# Autodesk Inventor assembly: FRCIntake2024
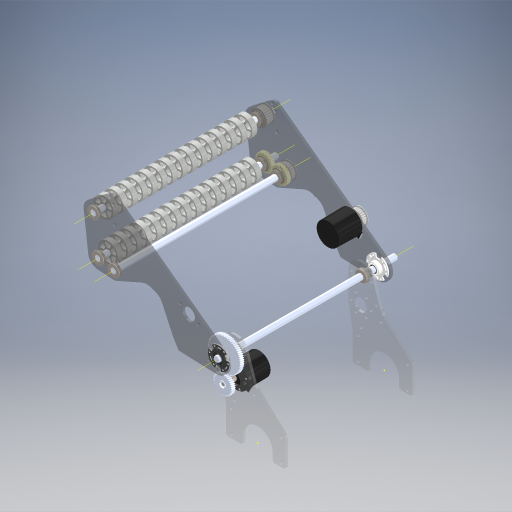
[picture p0: Inventor's stored thumbnail of the model, 512x512]
Saved by Autodesk Inventor 2024.2 (Build 282272000, 272)
## iProperties
Created: 2024-02-17
Part Number: FRCIntake2024
Document SubType Name: Assembly
Designer: rohan
Mass: 2142.23 g
Surface Area: 6813.45 cm^2
Volume: 1719.02 cm^3
Density: 1.24619 g/cm^3
Author: rohan
## Documents named in this file (14)
- C:\Users\rohan\OneDrive - Hillsborough County Public Schools\Robotics\FIRST-Robotics-Competition\Crescendo\Minotaur-Crescendo-Robot\FRCIntake2024.iam
- C:\Users\rohan\OneDrive - Hillsborough County Public Schools\Robotics\FIRST-Robotics-Competition\Crescendo\Minotaur-Crescendo-Robot\2D Overview - Part 2\wfsdf.ipt
- C:\Users\rohan\OneDrive - Hillsborough County Public Schools\Robotics\FIRST-Robotics-Competition\Crescendo\Minotaur-Crescendo-Robot\2D Overview - Part 2\cranking90s.ipt
- C:\Users\rohan\OneDrive - Hillsborough County Public Schools\Robotics\FIRST-Robotics-Competition\Crescendo\Minotaur-Crescendo-Robot\2D Overview - Part 2\am-2986 FR8ZZ Hex Bearing.ipt
- C:\Users\rohan\OneDrive - Hillsborough County Public Schools\Robotics\FIRST-Robotics-Competition\Crescendo\Minotaur-Crescendo-Robot\2D Overview - Part 2\1_2 Hex Bore Plastic VersaHub v2 (217-8079).iam
- C:\Users\rohan\OneDrive - Hillsborough County Public Schools\Robotics\FIRST-Robotics-Competition\Crescendo\Minotaur-Crescendo-Robot\2D Overview - Part 2\1_2 Acetal Spacer - 1_2 Hex (217-3261).ipt
- C:\Users\rohan\OneDrive - Hillsborough County Public Schools\Robotics\FIRST-Robotics-Competition\Crescendo\Minotaur-Crescendo-Robot\2D Overview - Part 2\1_2 OD Hex Stock (18) (217-3309).ipt
- C:\Users\rohan\Downloads\Minotaur-2024-CAD-main (2)\Minotaur-2024-CAD-main\Minotaur-2024-CAD-main\Minotaur-2024-CAD-main\64T Aluminum Spur Gear (20 DP, 1_2 Hex Bore) (217-3575)\64T Aluminum Spur Gear (20 DP, 1_.ipt
- C:\Users\rohan\Downloads\Minotaur-2024-CAD-main (2)\Minotaur-2024-CAD-main\Minotaur-2024-CAD-main\Minotaur-2024-CAD-main\Electronics\NEO-Brushless-Motor.ipt
- C:\Users\rohan\Downloads\36T Aluminum Spur Gear (20 DP, 1_2 Hex Bore) (217-3214)\36T Aluminum Spur Gear (20 DP, 1_2 Hex Bore) (217-3214).ipt
- C:\Users\rohan\OneDrive - Hillsborough County Public Schools\Robotics\FIRST-Robotics-Competition\Crescendo\Minotaur-Crescendo-Robot\2D Overview - Part 2\2 OD Straight Flex Wheel (217-6353).ipt
- C:\Users\rohan\OneDrive - Hillsborough County Public Schools\Robotics\FIRST-Robotics-Competition\Crescendo\Minotaur-Crescendo-Robot\2D Overview - Part 2\24t 15mm Wide 1_2_ Hex Bore Double Flange 5mm HTD Aluminum Pulley (217-4101).ipt
- C:\Users\rohan\OneDrive - Hillsborough County Public Schools\Robotics\FIRST-Robotics-Competition\Crescendo\Minotaur-Crescendo-Robot\2D Overview - Part 2\32t 20dp Aluminum 1_2_ Hex Bore Gear (217-5470).ipt
- C:\Users\rohan\OneDrive - Hillsborough County Public Schools\Robotics\FIRST-Robotics-Competition\Crescendo\Minotaur-Crescendo-Robot\2D Overview - Part 2\24t 9mm Wide 1_2_ Hex Bore Double Flange 5mm HTD Aluminum Pulley (217-3227).ipt
## Components (59 placed, 13 different names)
1. wfsdf:1 — Mate:1, Flush:1, Flush:2, Insert:2, Mate:8
2. wfsdf:2 — Mate:1, Flush:1, Flush:2, Insert:1, Mate:13, Mate:14
3. cranking90s:1 — Mate:11, Flush:3, Insert:8, Insert:9, Insert:10, Mate:16, Mate:20, Flush:7, Mate:26
4. cranking90s:2 — Mate:9, Mate:10, Flush:3, Insert:5, Insert:6, Insert:7, Mate:17, Mate:18, Mate:23, Mate:24
5. am-2986 FR8ZZ Hex Bearing:1 — Insert:2, Mate:2, Mate:6
6. am-2986 FR8ZZ Hex Bearing:2 — Insert:1, Mate:4
7. 1_2 Hex Bore Plastic VersaHub v2 (217-8079):1 [sub-assembly] — Mate:7, Mate:8, Mate:10
8. 1_2 Hex Bore Plastic VersaHub v2 (217-8079):2 [sub-assembly] — Mate:25, Mate:26
9. 1_2 Acetal Spacer - 1_2 Hex (217-3261):1 — Mate:3, Mate:4, Insert:3
10. 1_2 Acetal Spacer - 1_2 Hex (217-3261):2 — Mate:5, Mate:6
11. 1_2 OD Hex Stock (18) (217-3309):1 — Mate:2, Mate:3, Mate:5, Mate:7, Mate:9, Mate:11, Flush:7, Mate:25
12. 64T Aluminum Spur Gear (20 DP, 1_:1 — Insert:3
13. NEO-Brushless-Motor:1 — Mate:13, Mate:14, Insert:4
14. 36T Aluminum Spur Gear (20 DP, 1_2 Hex Bore) (217-3214):1 — Insert:4
15. am-2986 FR8ZZ Hex Bearing:3 — Insert:7, Insert:13
16. am-2986 FR8ZZ Hex Bearing:4 — Insert:10, Flush:5
17. am-2986 FR8ZZ Hex Bearing:5 — Insert:9, Flush:6, Mate:22
18. am-2986 FR8ZZ Hex Bearing:6 — Insert:6, Insert:12
19. am-2986 FR8ZZ Hex Bearing:7 — Insert:8, Flush:4
20. am-2986 FR8ZZ Hex Bearing:8 — Insert:5, Insert:11
21. 1_2 OD Hex Stock (18) (217-3309):2 — Mate:16, Flush:4, Mate:19
22. 1_2 OD Hex Stock (18) (217-3309):3 — Mate:17, Flush:5
23. 1_2 OD Hex Stock (18) (217-3309):4 — Mate:18, Flush:6, Mate:21
24. 24t 15mm Wide 1_2_ Hex Bore Double Flange 5mm HTD Aluminum Pulley (217-4101):1 — Insert:11
25. 32t 20dp Aluminum 1_2_ Hex Bore Gear (217-5470):1 — Insert:13, Insert:14
26. 32t 20dp Aluminum 1_2_ Hex Bore Gear (217-5470):2 — Insert:12
27. 24t 9mm Wide 1_2_ Hex Bore Double Flange 5mm HTD Aluminum Pulley (217-3227):1 — Insert:14
28. NEO-Brushless-Motor:2 — Mate:23, Mate:24, Insert:15
29. 24t 9mm Wide 1_2_ Hex Bore Double Flange 5mm HTD Aluminum Pulley (217-3227):2 — Insert:15
30. 2 OD Straight Flex Wheel (217-6353):1 — Mate:19, Mate:20
31. 2 OD Straight Flex Wheel (217-6353):2
32. 2 OD Straight Flex Wheel (217-6353):3
33. 2 OD Straight Flex Wheel (217-6353):4
34. 2 OD Straight Flex Wheel (217-6353):5
35. 2 OD Straight Flex Wheel (217-6353):6
36. 2 OD Straight Flex Wheel (217-6353):7
37. 2 OD Straight Flex Wheel (217-6353):8
38. 2 OD Straight Flex Wheel (217-6353):9
39. 2 OD Straight Flex Wheel (217-6353):10
40. 2 OD Straight Flex Wheel (217-6353):11
41. 2 OD Straight Flex Wheel (217-6353):12
42. 2 OD Straight Flex Wheel (217-6353):13
43. 2 OD Straight Flex Wheel (217-6353):14
44. 2 OD Straight Flex Wheel (217-6353):15
45. 2 OD Straight Flex Wheel (217-6353):16 — Mate:21, Mate:22
46. 2 OD Straight Flex Wheel (217-6353):17
47. 2 OD Straight Flex Wheel (217-6353):18
48. 2 OD Straight Flex Wheel (217-6353):19
49. 2 OD Straight Flex Wheel (217-6353):20
50. 2 OD Straight Flex Wheel (217-6353):21
51. 2 OD Straight Flex Wheel (217-6353):22
52. 2 OD Straight Flex Wheel (217-6353):23
53. 2 OD Straight Flex Wheel (217-6353):24
54. 2 OD Straight Flex Wheel (217-6353):25
55. 2 OD Straight Flex Wheel (217-6353):26
56. 2 OD Straight Flex Wheel (217-6353):27
57. 2 OD Straight Flex Wheel (217-6353):28
58. 2 OD Straight Flex Wheel (217-6353):29
59. 2 OD Straight Flex Wheel (217-6353):30
## Component patterns: (15 elements, first: 2 OD Straight Flex Wheel (217-6353):1), (15 elements, first: 2 OD Straight Flex Wheel (217-6353):16)
## Relationships (46: Mate 24, Insert 15, Flush 7)
- Mate:1 (317.5 mm): wfsdf:1 ↔ wfsdf:2
- Flush:1: wfsdf:1 ↔ wfsdf:2
- Flush:2: wfsdf:1 ↔ wfsdf:2
- Insert:1: wfsdf:2 ↔ am-2986 FR8ZZ Hex Bearing:2
- Insert:2: wfsdf:1 ↔ am-2986 FR8ZZ Hex Bearing:1
- Mate:2: am-2986 FR8ZZ Hex Bearing:1 ↔ 1_2 OD Hex Stock (18) (217-3309):1
- Mate:3: 1_2 Acetal Spacer - 1_2 Hex (217-3261):1 ↔ 1_2 OD Hex Stock (18) (217-3309):1
- Mate:4: am-2986 FR8ZZ Hex Bearing:2 ↔ 1_2 Acetal Spacer - 1_2 Hex (217-3261):1
- Mate:5: 1_2 Acetal Spacer - 1_2 Hex (217-3261):2 ↔ 1_2 OD Hex Stock (18) (217-3309):1
- Mate:6: am-2986 FR8ZZ Hex Bearing:1 ↔ 1_2 Acetal Spacer - 1_2 Hex (217-3261):2
- Insert:3: 1_2 Acetal Spacer - 1_2 Hex (217-3261):1 ↔ 64T Aluminum Spur Gear (20 DP, 1_:1
- Mate:7: 1_2 Hex Bore Plastic VersaHub v2 (217-8079):1 ↔ 1_2 OD Hex Stock (18) (217-3309):1
- Mate:8 (25.4762 mm): wfsdf:1 ↔ 1_2 Hex Bore Plastic VersaHub v2 (217-8079):1
- Mate:9: cranking90s:2 ↔ 1_2 OD Hex Stock (18) (217-3309):1
- Mate:10: cranking90s:2 ↔ 1_2 Hex Bore Plastic VersaHub v2 (217-8079):1
- Mate:11: cranking90s:1 ↔ 1_2 OD Hex Stock (18) (217-3309):1
- Mate:13: wfsdf:2 ↔ NEO-Brushless-Motor:1
- Mate:14: wfsdf:2 ↔ NEO-Brushless-Motor:1
- Insert:4: NEO-Brushless-Motor:1 ↔ 36T Aluminum Spur Gear (20 DP, 1_2 Hex Bore) (217-3214):1
- Flush:3: cranking90s:1 ↔ cranking90s:2
- Insert:5: cranking90s:2 ↔ am-2986 FR8ZZ Hex Bearing:8
- Insert:6: cranking90s:2 ↔ am-2986 FR8ZZ Hex Bearing:6
- Insert:7: cranking90s:2 ↔ am-2986 FR8ZZ Hex Bearing:3
- Insert:8: cranking90s:1 ↔ am-2986 FR8ZZ Hex Bearing:7
- Insert:9: cranking90s:1 ↔ am-2986 FR8ZZ Hex Bearing:5
- Insert:10: cranking90s:1 ↔ am-2986 FR8ZZ Hex Bearing:4
- Mate:16: cranking90s:1 ↔ 1_2 OD Hex Stock (18) (217-3309):2
- Mate:17: cranking90s:2 ↔ 1_2 OD Hex Stock (18) (217-3309):3
- Mate:18: cranking90s:2 ↔ 1_2 OD Hex Stock (18) (217-3309):4
- Flush:4: am-2986 FR8ZZ Hex Bearing:7 ↔ 1_2 OD Hex Stock (18) (217-3309):2
- Flush:5: am-2986 FR8ZZ Hex Bearing:4 ↔ 1_2 OD Hex Stock (18) (217-3309):3
- Flush:6: am-2986 FR8ZZ Hex Bearing:5 ↔ 1_2 OD Hex Stock (18) (217-3309):4
- Mate:19: 1_2 OD Hex Stock (18) (217-3309):2 ↔ 2 OD Straight Flex Wheel (217-6353):1
- Mate:20 (19.05 mm): cranking90s:1 ↔ 2 OD Straight Flex Wheel (217-6353):1
- Mate:21: 1_2 OD Hex Stock (18) (217-3309):4 ↔ 2 OD Straight Flex Wheel (217-6353):16
- Mate:22 (19.05 mm): am-2986 FR8ZZ Hex Bearing:5 ↔ 2 OD Straight Flex Wheel (217-6353):16
- Insert:11: am-2986 FR8ZZ Hex Bearing:8 ↔ 24t 15mm Wide 1_2_ Hex Bore Double Flange 5mm HTD Aluminum Pulley (217-4101):1
- Insert:12: am-2986 FR8ZZ Hex Bearing:6 ↔ 32t 20dp Aluminum 1_2_ Hex Bore Gear (217-5470):2
- Insert:13: am-2986 FR8ZZ Hex Bearing:3 ↔ 32t 20dp Aluminum 1_2_ Hex Bore Gear (217-5470):1
- Insert:14: 32t 20dp Aluminum 1_2_ Hex Bore Gear (217-5470):1 ↔ 24t 9mm Wide 1_2_ Hex Bore Double Flange 5mm HTD Aluminum Pulley (217-3227):1
- Mate:23: cranking90s:2 ↔ NEO-Brushless-Motor:2
- Mate:24: cranking90s:2 ↔ NEO-Brushless-Motor:2
- Insert:15: NEO-Brushless-Motor:2 ↔ 24t 9mm Wide 1_2_ Hex Bore Double Flange 5mm HTD Aluminum Pulley (217-3227):2
- Flush:7: cranking90s:1 ↔ 1_2 OD Hex Stock (18) (217-3309):1
- Mate:25: 1_2 Hex Bore Plastic VersaHub v2 (217-8079):2 ↔ 1_2 OD Hex Stock (18) (217-3309):1
- Mate:26: cranking90s:1 ↔ 1_2 Hex Bore Plastic VersaHub v2 (217-8079):2
